# Autodesk Inventor assembly: LCD
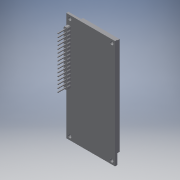
[picture p0: Inventor's stored thumbnail of the model, 180x180]
Saved by Autodesk Inventor 2016 (Build 200138000, 138)
## iProperties
Created: 2016-04-16
Part Number: LCD
Document SubType Name: Assembly
Designer: Jarrett
Author: Jarrett
## Documents named in this file (5)
- C:\Users\Jarrett\Dropbox (Personal)\Ergo Systems\Projects\yarndyer\CAD\LCD\LCD.iam
- C:\Users\Jarrett\Dropbox (Personal)\Ergo Systems\Projects\yarndyer\CAD\LCD\PCB.ipt
- C:\Users\Jarrett\Dropbox (Personal)\Ergo Systems\Projects\yarndyer\CAD\LCD\LCD Module.ipt
- C:\Users\Jarrett\Dropbox (Personal)\Ergo Systems\Projects\yarndyer\CAD\LCD\Pin Shroud.ipt
- C:\Users\Jarrett\Dropbox (Personal)\Ergo Systems\Projects\yarndyer\CAD\LCD\Pin.ipt
## Components (34 placed, 4 different names)
1. PCB:1 — Mate:1, Flush:1, Flush:2, Mate:5
2. LCD Module:1 — Mate:1, Flush:1, Flush:2
3. Pin Shroud:1 — Mate:4, Mate:2, Flush:3, Mate:5
4. Pin:1 — Mate:4, Mate:2, Flush:3
5. Pin Shroud:2
6. Pin:2
7. Pin Shroud:3
8. Pin:3
9. Pin Shroud:4
10. Pin:4
11. Pin Shroud:5
12. Pin:5
13. Pin Shroud:6
14. Pin:6
15. Pin Shroud:7
16. Pin:7
17. Pin Shroud:8
18. Pin:8
19. Pin Shroud:9
20. Pin:9
21. Pin Shroud:10
22. Pin:10
23. Pin Shroud:11
24. Pin:11
25. Pin Shroud:12
26. Pin:12
27. Pin Shroud:13
28. Pin:13
29. Pin Shroud:14
30. Pin:14
31. Pin Shroud:15
32. Pin:15
33. Pin Shroud:16
34. Pin:16
## Component patterns: (16 elements, first: Pin Shroud:1 + Pin:1)
## Relationships (7: Mate 4, Flush 3)
- Mate:1: PCB:1 ↔ LCD Module:1
- Flush:1 (4.6 mm): PCB:1 ↔ LCD Module:1
- Flush:2 (4.2 mm): PCB:1 ↔ LCD Module:1
- Mate:4: Pin Shroud:1 ↔ Pin:1
- Mate:2: Pin Shroud:1 ↔ Pin:1
- Flush:3 (3.5 mm): Pin Shroud:1 ↔ Pin:1
- Mate:5: PCB:1 ↔ Pin Shroud:1
